# Autodesk Inventor assembly: SPM
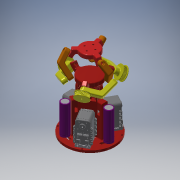
[picture p0: Inventor's stored thumbnail of the model, 180x180]
Saved by Autodesk Inventor 2019 (Build 230136000, 136)
## iProperties
Created: 2022-07-14
Part Number: SPM
Document SubType Name: Assembly
Designer: zreik
Author: zreik
## Documents named in this file (8)
- D:\Documents\HIAST\4th year\4th Year Project\Design\Current\SPM.iam
- D:\Documents\HIAST\4th year\4th Year Project\Design\Current\BottomPlatform.ipt
- D:\Documents\HIAST\4th year\4th Year Project\Design\Current\TopPlatform.ipt
- D:\Documents\HIAST\4th year\4th Year Project\Design\Current\Link1.ipt
- D:\Documents\HIAST\4th year\4th Year Project\Design\Current\Link2.ipt
- D:\Documents\HIAST\4th year\4th Year Project\Design\Current\MotorAssembled.iam
- D:\Documents\HIAST\4th year\4th Year Project\Design\Current\Battery.ipt
- Battery.ipt
## Components (14 placed, 6 different names)
1. BottomPlatform:1 — Mate:3, Mate:11, Mate:12, Mate:13, Angle:1, Angle:2, Mate:34, Mate:37, Mate:40, Mate:41, Mate:42, Mate:43, Mate:44, Mate:45, Mate:46, Mate:47
2. TopPlatform:1 — Mate:7, Mate:8, Mate:9, Mate:10, Angle:1, Mate:30, Mate:32, Mate:36
3. Link1:1 — Mate:3, Mate:5
4. Link2:1 — Mate:5, Mate:7, Mate:30
5. Link1:2 — Mate:33, Mate:34
6. Link2:2 — Mate:32, Mate:33
7. Link1:3 — Mate:35, Mate:37
8. Link2:3 — Mate:35, Mate:36
9. MotorAssembled:1 [sub-assembly] — Mate:40, Mate:41, Mate:42, Mate:43, Mate:44
10. MotorAssembled:2 [sub-assembly]
11. MotorAssembled:3 [sub-assembly]
12. Battery:1 — Mate:45, Mate:46, Mate:47
13. Battery:2
14. Battery:3
## Component patterns: (3 elements, first: MotorAssembled:1), (3 elements, first: Battery:1)
## Relationships (32: Mate 30, Angle 2)
- Mate:3: BottomPlatform:1 ↔ Link1:1
- Mate:5: Link1:1 ↔ Link2:1
- Mate:7: TopPlatform:1 ↔ Link2:1
- Mate:8: TopPlatform:1
- Mate:9: TopPlatform:1
- Mate:10: TopPlatform:1
- Mate:11: BottomPlatform:1
- Mate:12: BottomPlatform:1
- Mate:13: BottomPlatform:1
- Mate:14
- Mate:15
- Mate:16
- Mate:17
- Mate:27
- Angle:1 (0 deg): BottomPlatform:1 ↔ TopPlatform:1
- Mate:30: TopPlatform:1 ↔ Link2:1
- Mate:31
- Angle:2 (0 deg): BottomPlatform:1
- Mate:32: TopPlatform:1 ↔ Link2:2
- Mate:33: Link1:2 ↔ Link2:2
- Mate:34: BottomPlatform:1 ↔ Link1:2
- Mate:35: Link1:3 ↔ Link2:3
- Mate:36: TopPlatform:1 ↔ Link2:3
- Mate:37: BottomPlatform:1 ↔ Link1:3
- Mate:40: BottomPlatform:1 ↔ MotorAssembled:1
- Mate:41: BottomPlatform:1 ↔ MotorAssembled:1
- Mate:42: BottomPlatform:1 ↔ MotorAssembled:1
- Mate:43: BottomPlatform:1 ↔ MotorAssembled:1
- Mate:44: BottomPlatform:1 ↔ MotorAssembled:1
- Mate:45: BottomPlatform:1 ↔ Battery:1
- Mate:46 (9 mm): BottomPlatform:1 ↔ Battery:1
- Mate:47 (-6.7225 mm): BottomPlatform:1 ↔ Battery:1
